# Autodesk Inventor assembly: Assembly3
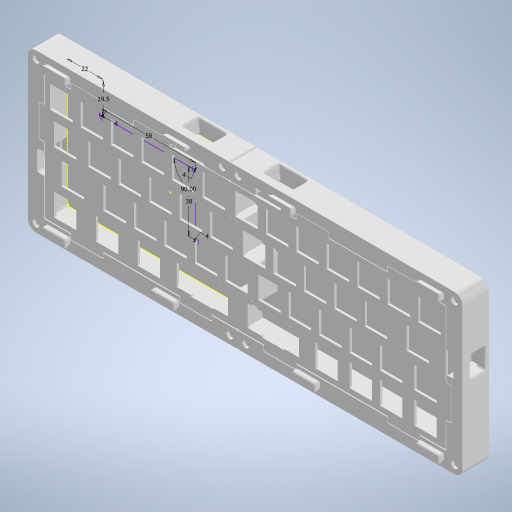
[picture p0: Inventor's stored thumbnail of the model, 512x512]
Saved by Autodesk Inventor 2023 (Build 270158000, 158)
## iProperties
Created: 2022-11-13
Part Number: Assembly3
Document SubType Name: Assembly
Designer: reide
Author: reide
## Documents named in this file (9)
- C:\Users\reide\OneDrive\Documents\Inventor\Fourier Keyboared Case\Assembly3.iam
- C:\Users\reide\OneDrive\Documents\Inventor\Fourier Keyboared Case\Plate_Left.ipt
- C:\Users\reide\OneDrive\Documents\Inventor\Fourier Keyboared Case\Plate_Right.ipt
- C:\Users\reide\OneDrive\Documents\Inventor\Fourier Keyboared Case\Mid_Left.ipt
- C:\Users\reide\OneDrive\Documents\Inventor\Fourier Keyboared Case\Top_Left.ipt
- C:\Users\reide\OneDrive\Documents\Inventor\Fourier Keyboared Case\BottomInner_left.ipt
- C:\Users\reide\OneDrive\Documents\Inventor\Fourier Keyboared Case\Mid_Right.ipt
- C:\Users\reide\OneDrive\Documents\Inventor\Fourier Keyboared Case\Top_Right.ipt
- C:\Users\reide\OneDrive\Documents\Inventor\Fourier Keyboared Case\BottomInner_right.ipt
## Components (8 placed, 8 different names)
1. Mid_Left:2 — Mate:3, Mate:4, Mate:5, Flush:1, Flush:2, Mate:6, Flush:3, Mate:10, Flush:4
2. Top_Left:2 — Flush:1, Flush:2, Mate:6
3. Plate_Left:2 — Mate:3, Mate:4, Mate:5, Flush:5
4. BottomInner_left:1 — Flush:3
5. Mid_Right:1 — Mate:7, Mate:8, Mate:9, Mate:10, Flush:4, Flush:6, Flush:7, Mate:11, Flush:8
6. Plate_Right:2 — Mate:7, Mate:8, Mate:9, Flush:5
7. Top_Right:3 — Flush:6, Flush:7, Mate:11
8. BottomInner_right:1 — Flush:8
## Relationships (17: Mate 9, Flush 8)
- Mate:3: Mid_Left:2 ↔ Plate_Left:2
- Mate:4 (0.3 mm): Mid_Left:2 ↔ Plate_Left:2
- Mate:5 (0.3 mm): Mid_Left:2 ↔ Plate_Left:2
- Flush:1: Mid_Left:2 ↔ Top_Left:2
- Flush:2: Mid_Left:2 ↔ Top_Left:2
- Mate:6: Mid_Left:2 ↔ Top_Left:2
- Flush:3: Mid_Left:2 ↔ BottomInner_left:1
- Mate:7: Mid_Right:1 ↔ Plate_Right:2
- Mate:8 (0.3 mm): Mid_Right:1 ↔ Plate_Right:2
- Mate:9 (0.3 mm): Mid_Right:1 ↔ Plate_Right:2
- Mate:10: Mid_Left:2 ↔ Mid_Right:1
- Flush:4: Mid_Left:2 ↔ Mid_Right:1
- Flush:5: Plate_Left:2 ↔ Plate_Right:2
- Flush:6: Mid_Right:1 ↔ Top_Right:3
- Flush:7: Mid_Right:1 ↔ Top_Right:3
- Mate:11: Mid_Right:1 ↔ Top_Right:3
- Flush:8: Mid_Right:1 ↔ BottomInner_right:1
